# Autodesk Inventor assembly: カート
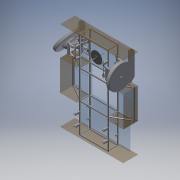
[picture p0: Inventor's stored thumbnail of the model, 180x180]
Saved by Autodesk Inventor 2018 (Build 220112000, 112)
## iProperties
Created: 2017-10-07
Part Number: カート
Material: 一般
Document SubType Name: Assembly
Designer: Kosei
Author: Kosei
## Documents named in this file (19)
- D:\Works\RBBR\CAD\カート.iam
- D:\Works\RBBR\CAD\シャーシ\シャーシ.iam
- D:\Works\RBBR\CAD\サスペンション\上アーム(前).iam
- D:\Works\RBBR\CAD\汎用部品\シャフト12x300mm.ipt
- D:\Works\RBBR\CAD\サスペンション\下アーム(前後).iam
- D:\Works\RBBR\CAD\サスペンション\車軸受け(前,左).iam
- D:\Works\RBBR\CAD\汎用部品\シャフト10x230mm.ipt
- D:\Works\RBBR\CAD\サスペンション\スプリング\スプリング.iam
- D:\Works\RBBR\CAD\車輪\前輪.ipt
- D:\Works\RBBR\CAD\車輪\前輪シャフト.ipt
- D:\Works\RBBR\CAD\車輪\前輪シャフトワッシャー.ipt
- D:\Works\RBBR\CAD\サスペンション\車軸受け(前,右).iam
- D:\Works\RBBR\CAD\ステアリング\ロッド.iam
- D:\Works\RBBR\CAD\ステアリング\車輪側スプロケット.ipt
- D:\Works\RBBR\CAD\装飾(仮)\前後.ipt
- D:\Works\RBBR\CAD\装飾(仮)\左右.ipt
- D:\Works\RBBR\CAD\装飾(仮)\泥除け1.ipt
- D:\Works\RBBR\CAD\装飾(仮)\床板.ipt
- D:\Works\RBBR\CAD\装飾(仮)\泥除け2.ipt
## Components (37 placed, 18 different names)
1. シャーシ:1 [sub-assembly] — フラッシュ:2, フラッシュ:3, フラッシュ:4, 円柱状:1, フラッシュ:5, 円柱状:2, フラッシュ:6, 円柱状:3, フラッシュ:7, 円柱状:4, フラッシュ:8, メイト:1, メイト:2, メイト:3, メイト:4, フラッシュ:9, フラッシュ:10, メイト:5, フラッシュ:11, メイト:6, フラッシュ:12, 角度:3, メイト:7, フラッシュ:13, フラッシュ:14, メイト:8, フラッシュ:15, フラッシュ:16, メイト:9, フラッシュ:17, フラッシュ:18, メイト:10, フラッシュ:19, メイト:12, フラッシュ:25, メイト:15, メイト:21, メイト:24, メイト:25, メイト:27
2. 泥除け2:1 — メイト:29, メイト:30, メイト:35
3. 泥除け2:2 — メイト:32, メイト:33, メイト:34
4. シャフト12x300mm:1 — 円柱状:1, フラッシュ:5, 円柱状:5, 円柱状:11
5. シャフト12x300mm:3 — 円柱状:3, フラッシュ:7, 円柱状:7
6. シャフト10x230mm:1 — 円柱状:9, フラッシュ:9, 円柱状:12
7. 上アーム(前):1 [sub-assembly] — 円柱状:5, メイト:1, リジッド:1, 角度:4
8. 下アーム(前後):1 [sub-assembly] — 円柱状:7, メイト:3, リジッド:2, 円柱状:9
9. 車軸受け(前,左):1 [sub-assembly] — リジッド:1, リジッド:2, 回転:2, リジッド:9
10. スプリング:1 [sub-assembly] — 円柱状:11, 円柱状:12
11. 前輪:1 — 回転:1, リジッド:5, 角度:8
12. 前輪シャフト:1 — 回転:1
13. 前輪シャフトワッシャー:1 — リジッド:5, 回転:2
14. シャフト12x300mm:2 — 円柱状:2, フラッシュ:6, 円柱状:6, 円柱状:13
15. シャフト12x300mm:4 — 円柱状:4, フラッシュ:8, 円柱状:8
16. シャフト10x230mm:2 — フラッシュ:10, 円柱状:10, 円柱状:14
17. 上アーム(前):2 [sub-assembly] — 円柱状:6, メイト:2, リジッド:3, 角度:5
18. 下アーム(前後):2 [sub-assembly] — 円柱状:8, メイト:4, リジッド:4, 円柱状:10
19. 車軸受け(前,右):1 [sub-assembly] — リジッド:3, リジッド:4, 回転:3, リジッド:8
20. スプリング:2 [sub-assembly] — 円柱状:13, 円柱状:14
21. 前輪:2 — リジッド:6, リジッド:7
22. 前輪シャフト:2 — リジッド:6
23. 前輪シャフトワッシャー:2 — リジッド:7, 回転:3
24. ロッド:1 [sub-assembly] — リジッド:8, リジッド:12, 角度:6
25. ロッド:2 [sub-assembly] — リジッド:9, リジッド:13, 角度:7
26. 車輪側スプロケット:1 — 円柱状:15, フラッシュ:12, リジッド:12, リジッド:13, 角度:3, 角度:6, 角度:7
27. シャフト12x300mm:5 — メイト:5, フラッシュ:11, メイト:6, 円柱状:15
28. 前後:1 — メイト:7, フラッシュ:13, フラッシュ:14, メイト:19, メイト:29, メイト:32
29. 前後:2 — メイト:8, フラッシュ:15, フラッシュ:16, メイト:22
30. 左右:1 — メイト:9, フラッシュ:17, フラッシュ:18, フラッシュ:26, メイト:16, フラッシュ:27, フラッシュ:28, メイト:26
31. 左右:2 — メイト:10, フラッシュ:19, 角度:8, フラッシュ:23, フラッシュ:24, フラッシュ:25, メイト:14, メイト:20, メイト:23, メイト:28
32. 泥除け1:1 — メイト:27, フラッシュ:24, メイト:28, メイト:35
33. 泥除け1:2 — メイト:15, フラッシュ:26, メイト:16, メイト:34
34. 泥除け1:3 — メイト:12, フラッシュ:23, メイト:14
35. 泥除け1:4 — フラッシュ:27, メイト:25, フラッシュ:28, メイト:26
36. 床板:1 — メイト:22, メイト:23, メイト:24
37. 床板:2 — メイト:19, メイト:20, メイト:21, メイト:30, メイト:33
## Relationships (89: Mate 30, Flush 24, CylindricalJoint 15, WeldJoint 11, Angle 6, RevoluteJoint 3)
- フラッシュ:2 [Flush]: シャーシ:1
- フラッシュ:3 [Flush]: シャーシ:1
- フラッシュ:4 [Flush]: シャーシ:1
- 円柱状:1 [CylindricalJoint]: シャーシ:1 ↔ シャフト12x300mm:1
- フラッシュ:5 [Flush]: シャーシ:1 ↔ シャフト12x300mm:1
- 円柱状:2 [CylindricalJoint]: シャーシ:1 ↔ シャフト12x300mm:2
- フラッシュ:6 [Flush]: シャーシ:1 ↔ シャフト12x300mm:2
- 円柱状:3 [CylindricalJoint]: シャーシ:1 ↔ シャフト12x300mm:3
- フラッシュ:7 [Flush]: シャーシ:1 ↔ シャフト12x300mm:3
- 円柱状:4 [CylindricalJoint]: シャーシ:1 ↔ シャフト12x300mm:4
- フラッシュ:8 [Flush]: シャーシ:1 ↔ シャフト12x300mm:4
- 円柱状:5 [CylindricalJoint]: シャフト12x300mm:1 ↔ 上アーム(前):1
- メイト:1 [Mate]: シャーシ:1 ↔ 上アーム(前):1
- 円柱状:6 [CylindricalJoint]: シャフト12x300mm:2 ↔ 上アーム(前):2
- メイト:2 [Mate]: シャーシ:1 ↔ 上アーム(前):2
- 円柱状:7 [CylindricalJoint]: シャフト12x300mm:3 ↔ 下アーム(前後):1
- メイト:3 [Mate]: シャーシ:1 ↔ 下アーム(前後):1
- 円柱状:8 [CylindricalJoint]: シャフト12x300mm:4 ↔ 下アーム(前後):2
- メイト:4 [Mate]: シャーシ:1 ↔ 下アーム(前後):2
- リジッド:1 [WeldJoint]: 上アーム(前):1 ↔ 車軸受け(前,左):1
- リジッド:2 [WeldJoint]: 下アーム(前後):1 ↔ 車軸受け(前,左):1
- リジッド:3 [WeldJoint]: 上アーム(前):2 ↔ 車軸受け(前,右):1
- リジッド:4 [WeldJoint]: 下アーム(前後):2 ↔ 車軸受け(前,右):1
- 円柱状:9 [CylindricalJoint]: シャフト10x230mm:1 ↔ 下アーム(前後):1
- フラッシュ:9 [Flush]: シャーシ:1 ↔ シャフト10x230mm:1
- フラッシュ:10 [Flush]: シャーシ:1 ↔ シャフト10x230mm:2
- 円柱状:10 [CylindricalJoint]: シャフト10x230mm:2 ↔ 下アーム(前後):2
- 円柱状:11 [CylindricalJoint]: シャフト12x300mm:1 ↔ スプリング:1
- 円柱状:12 [CylindricalJoint]: シャフト10x230mm:1 ↔ スプリング:1
- 円柱状:13 [CylindricalJoint]: シャフト12x300mm:2 ↔ スプリング:2
- 円柱状:14 [CylindricalJoint]: シャフト10x230mm:2 ↔ スプリング:2
- 回転:1 [RevoluteJoint]: 前輪:1 ↔ 前輪シャフト:1
- リジッド:5 [WeldJoint]: 前輪:1 ↔ 前輪シャフトワッシャー:1
- 回転:2 [RevoluteJoint]: 車軸受け(前,左):1 ↔ 前輪シャフトワッシャー:1
- リジッド:6 [WeldJoint]: 前輪:2 ↔ 前輪シャフト:2
- リジッド:7 [WeldJoint]: 前輪:2 ↔ 前輪シャフトワッシャー:2
- 回転:3 [RevoluteJoint]: 車軸受け(前,右):1 ↔ 前輪シャフトワッシャー:2
- リジッド:8 [WeldJoint]: 車軸受け(前,右):1 ↔ ロッド:1
- リジッド:9 [WeldJoint]: 車軸受け(前,左):1 ↔ ロッド:2
- メイト:5 [Mate]: シャーシ:1 ↔ シャフト12x300mm:5
- フラッシュ:11 [Flush]: シャーシ:1 ↔ シャフト12x300mm:5
- メイト:6 [Mate]: シャーシ:1 ↔ シャフト12x300mm:5
- 円柱状:15 [CylindricalJoint]: 車輪側スプロケット:1 ↔ シャフト12x300mm:5
- フラッシュ:12 [Flush] (160 mm): シャーシ:1 ↔ 車輪側スプロケット:1
- リジッド:12 [WeldJoint]: ロッド:1 ↔ 車輪側スプロケット:1
- リジッド:13 [WeldJoint]: ロッド:2 ↔ 車輪側スプロケット:1
- 角度:3 [Angle] (0 deg): シャーシ:1 ↔ 車輪側スプロケット:1
- 角度:4 [Angle] (0 deg): 上アーム(前):1
- 角度:5 [Angle] (10 deg): 上アーム(前):2
- 角度:6 [Angle] (0 deg): ロッド:1 ↔ 車輪側スプロケット:1
- 角度:7 [Angle] (0 deg): ロッド:2 ↔ 車輪側スプロケット:1
- メイト:7 [Mate]: シャーシ:1 ↔ 前後:1
- フラッシュ:13 [Flush] (40 mm): シャーシ:1 ↔ 前後:1
- フラッシュ:14 [Flush] (640 mm): シャーシ:1 ↔ 前後:1
- メイト:8 [Mate]: シャーシ:1 ↔ 前後:2
- フラッシュ:15 [Flush] (40 mm): シャーシ:1 ↔ 前後:2
- フラッシュ:16 [Flush] (640 mm): シャーシ:1 ↔ 前後:2
- メイト:9 [Mate]: シャーシ:1 ↔ 左右:1
- フラッシュ:17 [Flush] (40 mm): シャーシ:1 ↔ 左右:1
- フラッシュ:18 [Flush] (4 mm): シャーシ:1 ↔ 左右:1
- メイト:10 [Mate]: シャーシ:1 ↔ 左右:2
- フラッシュ:19 [Flush] (40 mm): シャーシ:1 ↔ 左右:2
- 角度:8 [Angle] (30 deg): 前輪:1 ↔ 左右:2
- メイト:12 [Mate]: シャーシ:1 ↔ 泥除け1:3
- フラッシュ:23 [Flush]: 左右:2 ↔ 泥除け1:3
- メイト:27 [Mate]: シャーシ:1 ↔ 泥除け1:1
- フラッシュ:24 [Flush]: 左右:2 ↔ 泥除け1:1
- フラッシュ:25 [Flush] (4 mm): シャーシ:1 ↔ 左右:2
- メイト:14 [Mate]: 左右:2 ↔ 泥除け1:3
- メイト:15 [Mate]: シャーシ:1 ↔ 泥除け1:2
- フラッシュ:26 [Flush]: 左右:1 ↔ 泥除け1:2
- メイト:16 [Mate]: 左右:1 ↔ 泥除け1:2
- フラッシュ:27 [Flush]: 左右:1 ↔ 泥除け1:4
- メイト:19 [Mate]: 前後:1 ↔ 床板:2
- メイト:20 [Mate]: 左右:2 ↔ 床板:2
- メイト:21 [Mate]: シャーシ:1 ↔ 床板:2
- メイト:22 [Mate]: 前後:2 ↔ 床板:1
- メイト:23 [Mate]: 左右:2 ↔ 床板:1
- メイト:24 [Mate]: シャーシ:1 ↔ 床板:1
- メイト:25 [Mate]: シャーシ:1 ↔ 泥除け1:4
- フラッシュ:28 [Flush]: 左右:1 ↔ 泥除け1:4
- メイト:26 [Mate]: 左右:1 ↔ 泥除け1:4
- メイト:28 [Mate]: 左右:2 ↔ 泥除け1:1
- メイト:29 [Mate]: 泥除け2:1 ↔ 前後:1
- メイト:30 [Mate]: 泥除け2:1 ↔ 床板:2
- メイト:32 [Mate]: 泥除け2:2 ↔ 前後:1
- メイト:33 [Mate]: 泥除け2:2 ↔ 床板:2
- メイト:34 [Mate]: 泥除け2:2 ↔ 泥除け1:2
- メイト:35 [Mate]: 泥除け2:1 ↔ 泥除け1:1
